# Autodesk Inventor assembly: Top Crossbrace
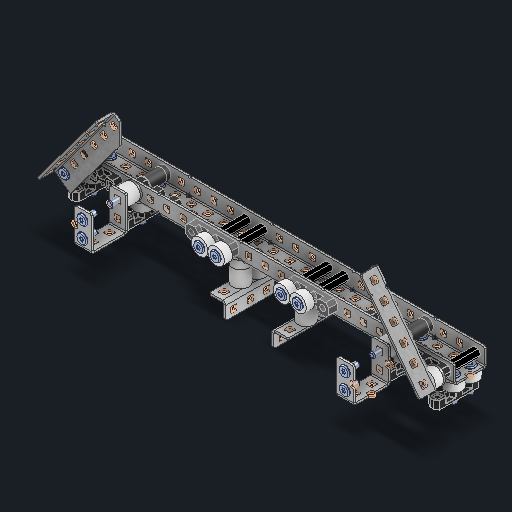
[picture p0: Inventor's stored thumbnail of the model, 512x512]
Saved by Autodesk Inventor 2025.1 (Build 291241000, 241)
## iProperties
Created: 2024-10-20
Part Number: Top Crossbrace
Document SubType Name: Assembly
Designer: Averey Ku
Author: Averey Ku
## Documents named in this file (29)
- C:\Users\avere\VEX\High Stakes\CAD\V2\Chassis\Structure\Top Crossbrace.iam
- C:\Users\avere\VEX\High Stakes\CAD\ROBOPROS-CAD-Inventor\Structure\C Channel\Aluminum 1x2x1\Alu C 1x2x1x17.ipt
- C:\Users\avere\VEX\High Stakes\CAD\ROBOPROS-CAD-Inventor\Structure\C Channel\Aluminum 2x2x2\Alu C 2x2x2x1.ipt
- C:\Users\avere\VEX\High Stakes\CAD\ROBOPROS-CAD-Inventor\Motion\Spacers\Spacer Nylon .500 OD\NSpacer White .500 OD x .375.ipt
- C:\Users\avere\VEX\High Stakes\CAD\ROBOPROS-CAD-Inventor\Motion\Shaft LS\Bearing Flat Low Profile.ipt
- C:\Users\avere\VEX\High Stakes\CAD\ROBOPROS-CAD-Inventor\Motion\Spacers\Washer Steel\SWasher .500 OD x .062500\SWasher .500 OD x .062500.ipt
- C:\Users\avere\VEX\High Stakes\CAD\ROBOPROS-CAD-Inventor\Motion\Spacers\Spacer Nylon .375 OD\NSpacer .375 OD x .125.ipt
- C:\Users\avere\VEX\High Stakes\CAD\ROBOPROS-CAD-Inventor\Motion\Spacers\Spacer Nylon .375 OD\NSpacer .375 OD x .500.ipt
- C:\Users\avere\VEX\High Stakes\CAD\ROBOPROS-CAD-Inventor\Structure\Hardware\Screw Steel - Star\SScrew Star Smooth 1.750.ipt
- C:\Users\avere\VEX\High Stakes\CAD\ROBOPROS-CAD-Inventor\Structure\Hardware\Screw Shoulder Robosource\SScrew Shoulder Smooth .375 x .12.ipt
- C:\Users\avere\VEX\High Stakes\CAD\ROBOPROS-CAD-Inventor\Motion\Spacers\Spacer Nylon .500 OD\NSpacer White .500 OD x .250.ipt
- C:\Users\avere\VEX\High Stakes\CAD\ROBOPROS-CAD-Inventor\Structure\Hardware\Screw Steel - Star\SScrew Star Smooth .750.ipt
- C:\Users\avere\VEX\High Stakes\CAD\ROBOPROS-CAD-Inventor\Structure\C Channel\Aluminum 1x2x1\Alu C 1x2x1x23.ipt
- C:\Users\avere\VEX\High Stakes\CAD\ROBOPROS-CAD-Inventor\Structure\Standoff\Standoff .875.ipt
- C:\Users\avere\VEX\High Stakes\CAD\ROBOPROS-CAD-Inventor\Structure\C Channel\Aluminum 1x3x1 Half Thick Cut\Alu C Half Thick 1x3x1x6.ipt
- C:\Users\avere\VEX\High Stakes\CAD\ROBOPROS-CAD-Inventor\Structure\Hardware\Screw Steel - Star\SScrew Star Smooth .875.ipt
- C:\Users\avere\VEX\High Stakes\CAD\ROBOPROS-CAD-Inventor\Structure\Hardware\Screw Steel - Star\SScrew Star Smooth .290.ipt
- C:\Users\avere\VEX\High Stakes\CAD\V2\Chassis\Structure\Right\Alu C 2x2x2x1 Right.ipt
- C:\Users\avere\VEX\High Stakes\CAD\V2\Chassis\Structure\Right\Bearing Flat Low Profile Right.ipt
- C:\Users\avere\VEX\High Stakes\CAD\V2\Chassis\Structure\Right\Alu C Half Thick 1x3x1x6 Right.ipt
- C:\Users\avere\VEX\High Stakes\CAD\ROBOPROS-CAD-Inventor\Motion\Spacers\Spacer Nylon .500 OD.ipt
- C:\Users\avere\VEX\High Stakes\CAD\ROBOPROS-CAD-Inventor\Motion\Spacers\Washer Steel\SWasher .500 OD x .062500.ipt
- C:\Users\avere\VEX\High Stakes\CAD\ROBOPROS-CAD-Inventor\Motion\Spacers\Spacer Nylon .375 OD.ipt
- C:\Users\avere\VEX\High Stakes\CAD\ROBOPROS-CAD-Inventor\Structure\Hardware\Screw Steel - Star.ipt
- C:\Users\avere\VEX\High Stakes\CAD\ROBOPROS-CAD-Inventor\Structure\Hardware\Screw Shoulder Robosource.ipt
- C:\Users\avere\VEX\High Stakes\CAD\ROBOPROS-CAD-Inventor\Structure\Standoff.ipt
- C:\Users\avere\VEX\High Stakes\CAD\ROBOPROS-CAD-Inventor\Motion\Spacers\Spacer Nylon .500 OD\NSpacer White .500 OD x .500.ipt
- C:\Users\avere\VEX\High Stakes\CAD\ROBOPROS-CAD-Inventor\Structure\Angle\Aluminum 1x1\Alu Angle 1x1x3.ipt
- C:\Users\avere\VEX\High Stakes\CAD\ROBOPROS-CAD-Inventor\Motion\Shaft LS\Bearing Flat.ipt
## Components (78 placed, 22 different names)
1. Alu C 1x2x1x23:1 — Insert:23, Flush:2, Insert:28, Insert:29, Insert:30, Insert:32, Insert:33, Insert:34, Mate:6, Insert:39, Insert:40, Insert:51, Insert:58, Mate:8, Insert:60, Insert:62, Insert:70, Insert:71, Insert:73, Insert:74, Insert:79, Mate:12, Insert:80, Mate:13
2. Alu C 1x2x1x17:1 — Insert:3, Insert:5, Mate:2, Insert:15, Flush:1, Flush:2
3. NSpacer White .500 OD x .250:21 — Insert:54
4. NSpacer White .500 OD x .500:22 — Insert:54, Mate:8, Insert:64
5. NSpacer White .500 OD x .250:23 — Insert:58
6. NSpacer White .500 OD x .500:24 — Mate:10
7. NSpacer White .500 OD x .250:25 — Insert:60
8. NSpacer White .500 OD x .500:26 — Insert:63
9. Alu Angle 1x1x3:1 — Insert:63, Mate:9
10. NSpacer White .500 OD x .250:27 — Insert:62
11. NSpacer White .500 OD x .500:28 — Mate:9
12. Alu Angle 1x1x3:2 — Insert:64, Mate:10
13. Standoff .875:3 — Insert:71
14. Standoff .875:4 — Insert:70
15. Bearing Flat:1 — Insert:77, Insert:78, Insert:80, Mate:13
16. Bearing Flat:2 — Insert:75, Insert:76, Insert:79
17. Standoff .875:5 — Insert:73
18. Standoff .875:6 — Insert:74
19. NSpacer White .500 OD x .250:29 — Insert:76, Insert:83
20. NSpacer White .500 OD x .250:30 — Insert:75, Mate:12, Insert:84
21. NSpacer White .500 OD x .250:31 — Insert:78, Insert:82
22. NSpacer White .500 OD x .250:32 — Insert:77, Insert:81
23. SScrew Star Smooth .750:23 — Insert:82
24. SScrew Star Smooth .750:24 — Insert:81
25. SScrew Star Smooth .750:25 — Insert:83
26. SScrew Star Smooth .750:26 — Insert:84
27. SScrew Shoulder Smooth .375 x .12:3 — Insert:52
28. Alu C 2x2x2x1:1 — Insert:2, Insert:16, Insert:52
29. NSpacer White .500 OD x .375:1 — Insert:2, Insert:4
30. Bearing Flat Low Profile:1 — Insert:3, Mate:2, Insert:12
31. SWasher .500 OD x .062500:1 — Insert:4, Insert:5, Insert:23
32. NSpacer .375 OD x .125:1 — Insert:11
33. NSpacer .375 OD x .500:2 — Insert:11, Insert:12
34. SScrew Star Smooth 1.750:1 — Insert:15
35. SScrew Shoulder Smooth .375 x .12:1 — Insert:16
36. Alu C Half Thick 1x3x1x6:1 — Insert:33, Insert:36, Insert:38
37. Bearing Flat Low Profile:8 — Insert:34, Mate:6, Insert:37
38. NSpacer White .500 OD x .250:14 — Insert:36
39. SWasher .500 OD x .062500:3 — Insert:37
40. SScrew Star Smooth .875:14 — Insert:38
41. Standoff .875:1 — Insert:39
42. SScrew Star Smooth .290:15 — Insert:40
43. SScrew Shoulder Smooth .375 x .12:4 — Insert:53
44. Alu C 2x2x2x1 Right:1 — Insert:41, Insert:45, Insert:53
45. NSpacer White .500 OD x .375:15 — Insert:41, Insert:42
46. Bearing Flat Low Profile Right:1 — Insert:43
47. SWasher .500 OD x .062500:4 — Insert:42
48. NSpacer .375 OD x .125:3 — Insert:44
49. NSpacer .375 OD x .500:4 — Insert:43, Insert:44
50. SScrew Star Smooth 1.750:16
51. SScrew Shoulder Smooth .375 x .12:2 — Insert:45
52. Alu C Half Thick 1x3x1x6 Right:1 — Insert:48, Insert:50
53. Bearing Flat Low Profile Right:3 — Insert:49
54. NSpacer White .500 OD x .250:18 — Insert:48
55. SWasher .500 OD x .062500:5 — Insert:49
56. SScrew Star Smooth .875:19 — Insert:50
57. Standoff .875:2
58. SScrew Star Smooth .290:20
59. NSpacer White .500 OD x .250:7 — Insert:32
60. NSpacer White .500 OD x .250:6 — Insert:30, Insert:31
61. Bearing Flat Low Profile:4 — Insert:31
62. SScrew Star Smooth .750:7 — Insert:29
63. SScrew Star Smooth .750:6 — Insert:28
64. NSpacer White .500 OD x .250:8
65. NSpacer White .500 OD x .250:9
66. Bearing Flat Low Profile:5
67. SScrew Star Smooth .750:8
68. SScrew Star Smooth .750:9
69. NSpacer White .500 OD x .250:16 — Insert:47, Insert:51
70. NSpacer White .500 OD x .250:17 — Insert:46, Mate:7
71. Bearing Flat Low Profile Right:2 — Insert:46, Insert:47
72. SScrew Star Smooth .750:17
73. SScrew Star Smooth .750:18 — Mate:7
74. NSpacer White .500 OD x .250:19
75. NSpacer White .500 OD x .250:20
76. Bearing Flat Low Profile Right:4
77. SScrew Star Smooth .750:21
78. SScrew Star Smooth .750:22
## Component patterns: Drivebay Attachments Left (2 elements), Drivebay Attachments Right (2 elements)
## Relationships (70: Insert 58, Mate 10, Flush 2)
- [Mate]: Alu C 1x2x1x17:1 ↔ Alu C 2x2x2x1:1
- Insert:2: Alu C 2x2x2x1:1 ↔ NSpacer White .500 OD x .375:1
- Insert:3: Alu C 1x2x1x17:1 ↔ Bearing Flat Low Profile:1
- Insert:4: NSpacer White .500 OD x .375:1 ↔ SWasher .500 OD x .062500:1
- Insert:5: Alu C 1x2x1x17:1 ↔ SWasher .500 OD x .062500:1
- Mate:2: Alu C 1x2x1x17:1 ↔ Bearing Flat Low Profile:1
- Insert:11: NSpacer .375 OD x .125:1 ↔ NSpacer .375 OD x .500:2
- Insert:12 (1.27 mm): Bearing Flat Low Profile:1 ↔ NSpacer .375 OD x .500:2
- Insert:15: Alu C 1x2x1x17:1 ↔ SScrew Star Smooth 1.750:1
- Insert:16: Alu C 2x2x2x1:1 ↔ SScrew Shoulder Smooth .375 x .12:1
- Flush:1 (-107.95 mm): Alu C 1x2x1x17:1
- Insert:23: Alu C 1x2x1x23:1 ↔ SWasher .500 OD x .062500:1
- Flush:2: Alu C 1x2x1x23:1 ↔ Alu C 1x2x1x17:1
- [Mate]: NSpacer White .500 OD x .250:6 ↔ Bearing Flat Low Profile:4
- [Insert] (1.27 mm): NSpacer White .500 OD x .250:7 ↔ Bearing Flat Low Profile:4
- Insert:28: Alu C 1x2x1x23:1 ↔ SScrew Star Smooth .750:6
- Insert:29: Alu C 1x2x1x23:1 ↔ SScrew Star Smooth .750:7
- Insert:30: Alu C 1x2x1x23:1 ↔ NSpacer White .500 OD x .250:6
- Insert:31 (1.27 mm): NSpacer White .500 OD x .250:6 ↔ Bearing Flat Low Profile:4
- Insert:32: Alu C 1x2x1x23:1 ↔ NSpacer White .500 OD x .250:7
- Insert:33 (14.2875 mm): Alu C 1x2x1x23:1 ↔ Alu C Half Thick 1x3x1x6:1
- Insert:34: Alu C 1x2x1x23:1 ↔ Bearing Flat Low Profile:8
- Mate:6: Alu C 1x2x1x23:1 ↔ Bearing Flat Low Profile:8
- Insert:36: Alu C Half Thick 1x3x1x6:1 ↔ NSpacer White .500 OD x .250:14
- Insert:37 (1.27 mm): Bearing Flat Low Profile:8 ↔ SWasher .500 OD x .062500:3
- Insert:38: Alu C Half Thick 1x3x1x6:1 ↔ SScrew Star Smooth .875:14
- Insert:39: Alu C 1x2x1x23:1 ↔ Standoff .875:1
- Insert:40: Alu C 1x2x1x23:1 ↔ SScrew Star Smooth .290:15
- Insert:41: Alu C 2x2x2x1 Right:1 ↔ NSpacer White .500 OD x .375:15
- Insert:42: NSpacer White .500 OD x .375:15 ↔ SWasher .500 OD x .062500:4
- Insert:43 (1.27 mm): Bearing Flat Low Profile Right:1 ↔ NSpacer .375 OD x .500:4
- Insert:44: NSpacer .375 OD x .125:3 ↔ NSpacer .375 OD x .500:4
- Insert:45: Alu C 2x2x2x1 Right:1 ↔ SScrew Shoulder Smooth .375 x .12:2
- Insert:46 (1.27 mm): NSpacer White .500 OD x .250:17 ↔ Bearing Flat Low Profile Right:2
- Insert:47 (1.27 mm): NSpacer White .500 OD x .250:16 ↔ Bearing Flat Low Profile Right:2
- Insert:48: Alu C Half Thick 1x3x1x6 Right:1 ↔ NSpacer White .500 OD x .250:18
- Insert:49 (1.27 mm): Bearing Flat Low Profile Right:3 ↔ SWasher .500 OD x .062500:5
- Insert:50: Alu C Half Thick 1x3x1x6 Right:1 ↔ SScrew Star Smooth .875:19
- Insert:51: Alu C 1x2x1x23:1 ↔ NSpacer White .500 OD x .250:16
- Mate:7: NSpacer White .500 OD x .250:17 ↔ SScrew Star Smooth .750:18
- Insert:52: SScrew Shoulder Smooth .375 x .12:3 ↔ Alu C 2x2x2x1:1
- Insert:53: SScrew Shoulder Smooth .375 x .12:4 ↔ Alu C 2x2x2x1 Right:1
- Insert:54: NSpacer White .500 OD x .250:21 ↔ NSpacer White .500 OD x .500:22
- [Insert]: NSpacer White .500 OD x .250:23 ↔ NSpacer White .500 OD x .500:24
- Insert:58: Alu C 1x2x1x23:1 ↔ NSpacer White .500 OD x .250:23
- Mate:8: Alu C 1x2x1x23:1 ↔ NSpacer White .500 OD x .500:22
- [Insert]: NSpacer White .500 OD x .250:25 ↔ NSpacer White .500 OD x .500:26
- Insert:60: Alu C 1x2x1x23:1 ↔ NSpacer White .500 OD x .250:25
- [Insert]: NSpacer White .500 OD x .250:27 ↔ NSpacer White .500 OD x .500:28
- Insert:62: Alu C 1x2x1x23:1 ↔ NSpacer White .500 OD x .250:27
- Insert:63: NSpacer White .500 OD x .500:26 ↔ Alu Angle 1x1x3:1
- Mate:9: Alu Angle 1x1x3:1 ↔ NSpacer White .500 OD x .500:28
- Insert:64: NSpacer White .500 OD x .500:22 ↔ Alu Angle 1x1x3:2
- Mate:10: NSpacer White .500 OD x .500:24 ↔ Alu Angle 1x1x3:2
- Insert:70: Alu C 1x2x1x23:1 ↔ Standoff .875:4
- Insert:71: Alu C 1x2x1x23:1 ↔ Standoff .875:3
- Insert:73: Alu C 1x2x1x23:1 ↔ Standoff .875:5
- Insert:74: Alu C 1x2x1x23:1 ↔ Standoff .875:6
- Insert:75: Bearing Flat:2 ↔ NSpacer White .500 OD x .250:30
- Insert:76: Bearing Flat:2 ↔ NSpacer White .500 OD x .250:29
- Insert:77: Bearing Flat:1 ↔ NSpacer White .500 OD x .250:32
- Insert:78: Bearing Flat:1 ↔ NSpacer White .500 OD x .250:31
- Insert:79: Alu C 1x2x1x23:1 ↔ Bearing Flat:2
- Mate:12: Alu C 1x2x1x23:1 ↔ NSpacer White .500 OD x .250:30
- Insert:80: Alu C 1x2x1x23:1 ↔ Bearing Flat:1
- Mate:13: Alu C 1x2x1x23:1 ↔ Bearing Flat:1
- Insert:81: NSpacer White .500 OD x .250:32 ↔ SScrew Star Smooth .750:24
- Insert:82: NSpacer White .500 OD x .250:31 ↔ SScrew Star Smooth .750:23
- Insert:83: NSpacer White .500 OD x .250:29 ↔ SScrew Star Smooth .750:25
- Insert:84: NSpacer White .500 OD x .250:30 ↔ SScrew Star Smooth .750:26
## Named parameters: d46_d43 = 1.27 mm, d47_d31 = 0 mm, d96_d94 = 0 mm, d100_d94 = 0 mm, d102_d100_d94 = 0 mm
